# Autodesk Inventor assembly: Ensamble_6_Pinza
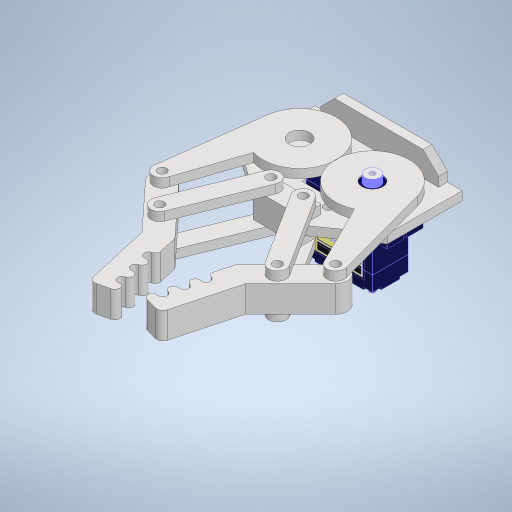
[picture p0: Inventor's stored thumbnail of the model, 512x512]
Saved by Autodesk Inventor 2023 (Build 270158000, 158)
## iProperties
Created: 2024-09-27
Part Number: Ensamble_6_Pinza
Document SubType Name: Assembly
Designer: sebas
Author: sebas
## Documents named in this file (6)
- C:\Users\sebas\OneDrive\Documentos\ILLERO_MODELADO_ROBOT\Ensamble_6_Pinza.iam
- C:\Users\sebas\OneDrive\Documentos\ILLERO_MODELADO_ROBOT\MicroServo-SG90.ipt
- C:\Users\sebas\OneDrive\Documentos\ILLERO_MODELADO_ROBOT\Pinza_pieza1.ipt
- C:\Users\sebas\OneDrive\Documentos\ILLERO_MODELADO_ROBOT\Pinza_pieza2.ipt
- C:\Users\sebas\OneDrive\Documentos\ILLERO_MODELADO_ROBOT\Pinza_pieza3.ipt
- C:\Users\sebas\OneDrive\Documentos\ILLERO_MODELADO_ROBOT\Pinza_pieza4.ipt
## Components (10 placed, 5 different names)
1. Pinza_pieza1:1 — Coincidencia:38, Coincidencia:39, Coincidencia:40, Coincidencia:41, Coincidencia:42, Coincidencia:43, Coincidencia:44, Coincidencia:45, Coincidencia:52, Coincidencia:59, Coincidencia:60, Coincidencia:62, Coincidencia:63, Coincidencia:65, Coincidencia:66, Coincidencia:67
2. Pinza_pieza2:1 — Coincidencia:38, Coincidencia:39, Coincidencia:48, Coincidencia:49
3. Pinza_pieza2:2 — Coincidencia:40, Coincidencia:41, Coincidencia:46, Coincidencia:47
4. Pinza_pieza2:3 — Coincidencia:42, Coincidencia:43, Coincidencia:58
5. Pinza_pieza2:4 — Coincidencia:44, Coincidencia:45, Coincidencia:50
6. Pinza_pieza3:2 — Coincidencia:46, Coincidencia:47, Coincidencia:50, Coincidencia:64
7. Pinza_pieza3:3 — Coincidencia:48, Coincidencia:49, Coincidencia:56, Coincidencia:57, Coincidencia:58
8. MicroServo-SG90:2 — Coincidencia:52, Coincidencia:59, Coincidencia:60, Coincidencia:61
9. Pinza_pieza4:1 — Coincidencia:56, Coincidencia:57, Coincidencia:61
10. Pinza_pieza4:2 — Coincidencia:62, Coincidencia:63, Coincidencia:64
## Relationships (26: Mate 26)
- Coincidencia:38 [Mate]: Pinza_pieza1:1 ↔ Pinza_pieza2:1
- Coincidencia:39 [Mate]: Pinza_pieza1:1 ↔ Pinza_pieza2:1
- Coincidencia:40 [Mate]: Pinza_pieza1:1 ↔ Pinza_pieza2:2
- Coincidencia:41 [Mate]: Pinza_pieza1:1 ↔ Pinza_pieza2:2
- Coincidencia:42 [Mate]: Pinza_pieza1:1 ↔ Pinza_pieza2:3
- Coincidencia:43 [Mate]: Pinza_pieza1:1 ↔ Pinza_pieza2:3
- Coincidencia:44 [Mate]: Pinza_pieza1:1 ↔ Pinza_pieza2:4
- Coincidencia:45 [Mate]: Pinza_pieza1:1 ↔ Pinza_pieza2:4
- Coincidencia:46 [Mate]: Pinza_pieza2:2 ↔ Pinza_pieza3:2
- Coincidencia:47 [Mate]: Pinza_pieza2:2 ↔ Pinza_pieza3:2
- Coincidencia:48 [Mate]: Pinza_pieza2:1 ↔ Pinza_pieza3:3
- Coincidencia:49 [Mate]: Pinza_pieza2:1 ↔ Pinza_pieza3:3
- Coincidencia:50 [Mate]: Pinza_pieza2:4 ↔ Pinza_pieza3:2
- Coincidencia:52 [Mate]: Pinza_pieza1:1 ↔ MicroServo-SG90:2
- Coincidencia:56 [Mate]: Pinza_pieza3:3 ↔ Pinza_pieza4:1
- Coincidencia:57 [Mate]: Pinza_pieza3:3 ↔ Pinza_pieza4:1
- Coincidencia:58 [Mate]: Pinza_pieza2:3 ↔ Pinza_pieza3:3
- Coincidencia:59 [Mate]: Pinza_pieza1:1 ↔ MicroServo-SG90:2
- Coincidencia:60 [Mate]: Pinza_pieza1:1 ↔ MicroServo-SG90:2
- Coincidencia:61 [Mate]: MicroServo-SG90:2 ↔ Pinza_pieza4:1
- Coincidencia:62 [Mate] (3 mm): Pinza_pieza1:1 ↔ Pinza_pieza4:2
- Coincidencia:63 [Mate]: Pinza_pieza1:1 ↔ Pinza_pieza4:2
- Coincidencia:64 [Mate]: Pinza_pieza3:2 ↔ Pinza_pieza4:2
- Coincidencia:65 [Mate]: Pinza_pieza1:1
- Coincidencia:66 [Mate]: Pinza_pieza1:1
- Coincidencia:67 [Mate]: Pinza_pieza1:1
